# Autodesk Inventor assembly: WheelIntake3.0
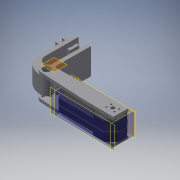
[picture p0: Inventor's stored thumbnail of the model, 180x180]
Saved by Autodesk Inventor 2017 (Build 210142000, 142)
## iProperties
Created: 2017-12-13
Part Number: WheelIntake3.0
Document SubType Name: Assembly
Designer: User
Author: User
## Documents named in this file (5)
- C:\Robotics\CAD\2017-18_CAD\WheelIntake3.0.iam
- C:\Robotics\CAD\2017-18_CAD\WheelIntakeMount3.0.ipt
- C:\Robotics\CAD\2017-18_CAD\WheelIntake3.0Tensioner.ipt
- C:\Robotics\CAD\2017-18_CAD\Prototypes\WheelIntakeBase3.0.ipt
- C:\Robotics\CAD\COTSParts\Rev\REV-41-1300.ipt
## Components (4 placed, 4 different names)
1. WheelIntakeMount3.0:1 — Insert:1, Insert:2, Insert:3
2. WheelIntake3.0Tensioner:1 — Mate:1, Flush:1, Mate:2
3. WheelIntakeBase3.0:1 — Insert:1, Mate:1, Flush:1, Mate:2
4. REV-41-1300:1 — Insert:2, Insert:3
## Relationships (6: Insert 3, Mate 2, Flush 1)
- Insert:1: WheelIntakeMount3.0:1 ↔ WheelIntakeBase3.0:1
- Mate:1: WheelIntake3.0Tensioner:1 ↔ WheelIntakeBase3.0:1
- Flush:1 (3.175 mm): WheelIntake3.0Tensioner:1 ↔ WheelIntakeBase3.0:1
- Mate:2: WheelIntake3.0Tensioner:1 ↔ WheelIntakeBase3.0:1
- Insert:2: WheelIntakeMount3.0:1 ↔ REV-41-1300:1
- Insert:3: WheelIntakeMount3.0:1 ↔ REV-41-1300:1
